# Autodesk Inventor assembly: 사각형 OV-PAM 10패턴
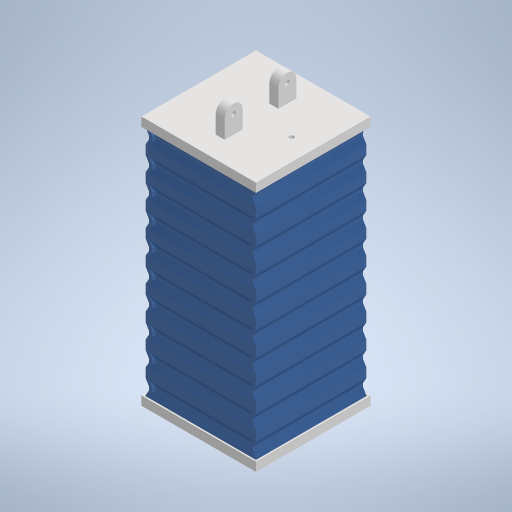
[picture p0: Inventor's stored thumbnail of the model, 512x512]
Saved by Autodesk Inventor 2024 (Build 280153000, 153)
## iProperties
Created: 2023-06-16
Part Number: 사각형 OV-PAM 10패턴
Document SubType Name: Assembly
Designer: jsw
Author: jsw
## Documents named in this file (5)
- C:\승원\co-op\OV-PAM\사각형 OV-PAM 10패턴.iam
- C:\승원\co-op\OV-PAM\사각형 OV-PAM 10패턴 층 중단 하단 연결 층.ipt
- C:\승원\co-op\OV-PAM\사각형 OV-PAM 10패턴 층 한개.ipt
- C:\승원\co-op\OV-PAM\사각형 OV-PAM 10패턴 상단.ipt
- C:\승원\co-op\OV-PAM\사각형 OV-PAM 10패턴 하단.ipt
## Components (12 placed, 4 different names)
1. 사각형 OV-PAM 10패턴 층 중단 하단 연결 층:1 — 메이트:1, 플러쉬:1, 플러쉬:4, 메이트:3, 메이트:5
2. 사각형 OV-PAM 10패턴 층 중단 하단 연결 층:2 — 메이트:2, 플러쉬:3, 플러쉬:5, 메이트:4, 메이트:6, 메이트:8, 메이트:9
3. 사각형 OV-PAM 10패턴 상단:1 — 메이트:3, 메이트:4, 메이트:5
4. 사각형 OV-PAM 10패턴 하단:1 — 메이트:6, 메이트:8, 메이트:9
5. 사각형 OV-PAM 10패턴 층 한개:1 — 메이트:1, 플러쉬:1, 플러쉬:4
6. 사각형 OV-PAM 10패턴 층 한개:2
7. 사각형 OV-PAM 10패턴 층 한개:3
8. 사각형 OV-PAM 10패턴 층 한개:4
9. 사각형 OV-PAM 10패턴 층 한개:5
10. 사각형 OV-PAM 10패턴 층 한개:6
11. 사각형 OV-PAM 10패턴 층 한개:7
12. 사각형 OV-PAM 10패턴 층 한개:8 — 메이트:2, 플러쉬:3, 플러쉬:5
## Component patterns: (8 elements, first: 사각형 OV-PAM 10패턴 층 한개:1)
## Relationships (12: Mate 8, Flush 4)
- 메이트:1 [Mate]: 사각형 OV-PAM 10패턴 층 중단 하단 연결 층:1 ↔ 사각형 OV-PAM 10패턴 층 한개:1
- 플러쉬:1 [Flush]: 사각형 OV-PAM 10패턴 층 중단 하단 연결 층:1 ↔ 사각형 OV-PAM 10패턴 층 한개:1
- 메이트:2 [Mate]: 사각형 OV-PAM 10패턴 층 중단 하단 연결 층:2 ↔ 사각형 OV-PAM 10패턴 층 한개:8
- 플러쉬:3 [Flush]: 사각형 OV-PAM 10패턴 층 중단 하단 연결 층:2 ↔ 사각형 OV-PAM 10패턴 층 한개:8
- 플러쉬:4 [Flush]: 사각형 OV-PAM 10패턴 층 중단 하단 연결 층:1 ↔ 사각형 OV-PAM 10패턴 층 한개:1
- 플러쉬:5 [Flush]: 사각형 OV-PAM 10패턴 층 중단 하단 연결 층:2 ↔ 사각형 OV-PAM 10패턴 층 한개:8
- 메이트:3 [Mate]: 사각형 OV-PAM 10패턴 층 중단 하단 연결 층:1 ↔ 사각형 OV-PAM 10패턴 상단:1
- 메이트:4 [Mate]: 사각형 OV-PAM 10패턴 층 중단 하단 연결 층:2 ↔ 사각형 OV-PAM 10패턴 상단:1
- 메이트:5 [Mate]: 사각형 OV-PAM 10패턴 층 중단 하단 연결 층:1 ↔ 사각형 OV-PAM 10패턴 상단:1
- 메이트:6 [Mate]: 사각형 OV-PAM 10패턴 층 중단 하단 연결 층:2 ↔ 사각형 OV-PAM 10패턴 하단:1
- 메이트:8 [Mate]: 사각형 OV-PAM 10패턴 층 중단 하단 연결 층:2 ↔ 사각형 OV-PAM 10패턴 하단:1
- 메이트:9 [Mate]: 사각형 OV-PAM 10패턴 층 중단 하단 연결 층:2 ↔ 사각형 OV-PAM 10패턴 하단:1
